# Autodesk Inventor assembly: parachute_structure_asm
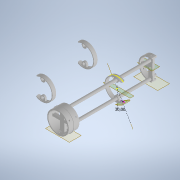
[picture p0: Inventor's stored thumbnail of the model, 180x180]
Saved by Autodesk Inventor 2020 (Build 240168000, 168)
## iProperties
Created: 2022-03-10
Part Number: parachute_structure_asm
Document SubType Name: Assembly
Designer: sp
Author: sp
## Documents named in this file (6)
- C:\Users\sp\Documents\Rocket\rocket\CAD\parachute_structure_asm.iam
- C:\Users\sp\Documents\Rocket\rocket\CAD\stange.ipt
- C:\Users\sp\Documents\Rocket\rocket\CAD\Verbindungsring_2_2.ipt
- C:\Users\sp\Documents\Rocket\rocket\CAD\Verbindungsring_2_3.ipt
- C:\Users\sp\Documents\Rocket\rocket\CAD\Parachute_Verb.ipt
- C:\Users\sp\Documents\Rocket\rocket\CAD\Parachute_Verb_V2.ipt
## Components (7 placed, 5 different names)
1. stange:1 — Einfügen:1, Einfügen:3, Passend:2
2. stange:2 — Einfügen:2, Passend:1
3. Verbindungsring_2_2:1 — Einfügen:1, Einfügen:2
4. Verbindungsring_2_3:1 — Einfügen:3
5. Parachute_Verb:1 — Passend:1, Passend:2
6. Parachute_Verb_V2:1
7. Parachute_Verb_V2:2
## Relationships (5: Insert 3, Mate 2)
- Einfügen:1 [Insert]: stange:1 ↔ Verbindungsring_2_2:1
- Einfügen:2 [Insert]: stange:2 ↔ Verbindungsring_2_2:1
- Einfügen:3 [Insert]: stange:1 ↔ Verbindungsring_2_3:1
- Passend:1 [Mate]: stange:2 ↔ Parachute_Verb:1
- Passend:2 [Mate]: stange:1 ↔ Parachute_Verb:1
